# Autodesk Inventor assembly: 20171110 Zusammengesetzt
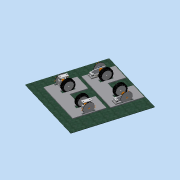
[picture p0: Inventor's stored thumbnail of the model, 180x180]
Saved by Autodesk Inventor 2015 (Build 190159000, 159)
## iProperties
Created: 2017-11-10
Part Number: 20171110 Zusammengesetzt
Document SubType Name: Assembly
Designer: Christoph Soppa
Author: Christoph Soppa
## Documents named in this file (18)
- C:\Users\Christoph Soppa\Desktop\THM Automatisierungs- technik\Sem. 8 Projektarbeit\Bauteile\20171110 Zusammengesetzt.iam
- C:\Users\Christoph Soppa\Desktop\THM Automatisierungs- technik\Sem. 8 Projektarbeit\Bauteile\O Ring 72x3,5x65.ipt
- C:\Users\Christoph Soppa\Desktop\THM Automatisierungs- technik\Sem. 8 Projektarbeit\Bauteile\Rad d72 b4 r3.5.ipt
- C:\Users\Christoph Soppa\Desktop\THM Automatisierungs- technik\Sem. 8 Projektarbeit\Bauteile\Drehgeber 2400 .ipt
- C:\Users\Christoph Soppa\Desktop\THM Automatisierungs- technik\Sem. 8 Projektarbeit\Bauteile\Boden.ipt
- C:\Users\Christoph Soppa\Desktop\THM Automatisierungs- technik\Sem. 8 Projektarbeit\Bauteile\FahrwerkbasisBsp.ipt
- C:\Users\Christoph Soppa\Desktop\THM Automatisierungs- technik\Sem. 8 Projektarbeit\Bauteile\Montageplatte.ipt
- C:\Users\Christoph Soppa\Desktop\THM Automatisierungs- technik\Sem. 8 Projektarbeit\Bauteile\Stehlager 6mm.ipt
- C:\Users\Christoph Soppa\Desktop\THM Automatisierungs- technik\Sem. 8 Projektarbeit\Bauteile\6mm Welle.ipt
- C:\Users\Christoph Soppa\Desktop\THM Automatisierungs- technik\Sem. 8 Projektarbeit\Bauteile\Kupplung.ipt
- C:\Users\Christoph Soppa\Desktop\THM Automatisierungs- technik\Sem. 8 Projektarbeit\Bauteile\Armrechts.ipt
- C:\Users\Christoph Soppa\Desktop\THM Automatisierungs- technik\Sem. 8 Projektarbeit\Bauteile\Armlinks.ipt
- C:\Users\Christoph Soppa\Desktop\THM Automatisierungs- technik\Sem. 8 Projektarbeit\Bauteile\Gummierung Antrieb.ipt
- C:\Users\Christoph Soppa\Desktop\THM Automatisierungs- technik\Sem. 8 Projektarbeit\Bauteile\Antriebsrad 80.ipt
- C:\Users\Christoph Soppa\Desktop\THM Automatisierungs- technik\Sem. 8 Projektarbeit\Bauteile\B Arm.ipt
- C:\Users\Christoph Soppa\Desktop\THM Automatisierungs- technik\Sem. 8 Projektarbeit\Bauteile\B Montageplatte.ipt
- C:\Users\Christoph Soppa\Desktop\THM Automatisierungs- technik\Sem. 8 Projektarbeit\Bauteile\B Oben.ipt
- C:\Users\Christoph Soppa\Desktop\THM Automatisierungs- technik\Sem. 8 Projektarbeit\Bauteile\Federführung.ipt
## Components (47 placed, 17 different names)
1. O Ring 72x3,5x65:1 — Passend:44, Passend:45
2. O Ring 72x3,5x65:2 — Passend:3, Passend:4
3. Rad d72 b4 r3.5:1 — Passend:3, Passend:4, Passend:10, Fluchtend:3, Passend:24, Passend:25, Passend:26
4. Rad d72 b4 r3.5:2 — Passend:40, Passend:41, Passend:42, Passend:45
5. Drehgeber 2400 :1 — Passend:36, Passend:37, Passend:38, Passend:39
6. Drehgeber 2400 :2 — Passend:20, Passend:21, Passend:22, Passend:23
7. Boden:1 — Passend:9, Passend:10, Fluchtend:3, Passend:12, Passend:46, Passend:49, Passend:53, Passend:55, Fluchtend:14, Passend:82, Passend:87, Passend:94, Passend:96
8. FahrwerkbasisBsp:1 — Passend:12, Passend:16, Passend:26, Passend:27, Passend:28, Passend:42, Passend:43, Passend:48, Passend:50, Passend:52, Passend:54
9. Montageplatte:1 — Passend:13, Fluchtend:5, Passend:14, Fluchtend:6, Fluchtend:7, Passend:16
10. Stehlager 6mm:1 — Passend:13, Fluchtend:5, Passend:19
11. Stehlager 6mm:2 — Passend:14, Fluchtend:6, Fluchtend:7, Fluchtend:8, Passend:15, Passend:17
12. 6mm Welle:1 — Fluchtend:8, Passend:15, Passend:18
13. Kupplung:1 — Passend:22, Passend:23, Passend:24, Passend:25, Passend:27
14. Armrechts:1 — Passend:17, Passend:18, Passend:19, Passend:20, Passend:21
15. Stehlager 6mm:3 — Passend:30, Passend:33, Passend:34, Passend:35, Fluchtend:11
16. Stehlager 6mm:4 — Passend:29, Fluchtend:9, Fluchtend:10, Passend:31, Passend:32
17. Montageplatte:2 — Passend:28, Passend:29, Passend:30, Fluchtend:9, Fluchtend:10
18. Armlinks:1 — Passend:31, Passend:32, Passend:33, Passend:34, Passend:36, Passend:37
19. Kupplung:2 — Passend:38, Passend:39, Passend:40, Passend:41, Passend:43, Passend:44, Passend:46
20. 6mm Welle:2 — Passend:35, Fluchtend:11
21. Gummierung Antrieb:1 — Passend:47, Fluchtend:12, Passend:49, Passend:50
22. Gummierung Antrieb:2 — Fluchtend:13, Passend:51, Passend:53, Passend:54
23. Antriebsrad 80:1 — Fluchtend:13, Passend:51, Passend:52
24. Antriebsrad 80:2 — Passend:47, Fluchtend:12, Passend:48
25. FahrwerkbasisBsp:2 — Passend:55, Fluchtend:14, Passend:80, Passend:81, Passend:83, Passend:84, Passend:85, Passend:86, Passend:92, Passend:93, Passend:95, Passend:97
26. B Arm:1 — Passend:67, Passend:68, Passend:71, Passend:72
27. B Montageplatte:1 — Passend:60, Passend:61, Fluchtend:18, Fluchtend:19, Passend:84
28. B Montageplatte:2 — Passend:62, Passend:63, Fluchtend:17, Fluchtend:20, Passend:80
29. B Arm:2 — Passend:66, Passend:69, Passend:70, Passend:73
30. B Oben:1 — Passend:64, Fluchtend:21
31. B Oben:2 — Passend:65, Fluchtend:22
32. Federführung:1 — Passend:63, Fluchtend:20, Passend:64, Fluchtend:21, Passend:67
33. Federführung:2 — Passend:61, Fluchtend:19, Passend:65, Fluchtend:22, Passend:66
34. Federführung:3 — Passend:60, Fluchtend:18, Passend:69
35. Federführung:4 — Passend:62, Fluchtend:17, Passend:68
36. Kupplung:3 — Passend:58, Passend:75, Passend:76, Passend:79, Passend:82, Passend:83
37. Kupplung:4 — Passend:59, Passend:74, Passend:77, Passend:78, Passend:86, Passend:87, Passend:90
38. Drehgeber 2400 :3 — Passend:71, Passend:72, Passend:75, Passend:79
39. Drehgeber 2400 :4 — Passend:70, Passend:73, Passend:74, Passend:78
40. Gummierung Antrieb:3 — Passend:57, Fluchtend:15
41. Gummierung Antrieb:4 — Passend:56, Fluchtend:16, Passend:97
42. O Ring 72x3,5x65:3 — Passend:90, Passend:91
43. O Ring 72x3,5x65:4 — Passend:88, Passend:89
44. Rad d72 b4 r3.5:3 — Passend:59, Passend:77, Passend:85, Passend:91
45. Rad d72 b4 r3.5:4 — Passend:58, Passend:76, Passend:81, Passend:88, Passend:89
46. Antriebsrad 80:3 — Passend:57, Fluchtend:15, Passend:92, Passend:93, Passend:94
47. Antriebsrad 80:4 — Passend:56, Fluchtend:16, Passend:95, Passend:96
## Relationships (109: Mate 90, Flush 19)
- Passend:3 [Mate]: O Ring 72x3,5x65:2 ↔ Rad d72 b4 r3.5:1
- Passend:4 [Mate]: O Ring 72x3,5x65:2 ↔ Rad d72 b4 r3.5:1
- Passend:9 [Mate]: Boden:1
- Passend:10 [Mate] (36 mm): Rad d72 b4 r3.5:1 ↔ Boden:1
- Fluchtend:3 [Flush] (100 mm): Rad d72 b4 r3.5:1 ↔ Boden:1
- Passend:12 [Mate] (5 mm): Boden:1 ↔ FahrwerkbasisBsp:1
- Passend:13 [Mate]: Montageplatte:1 ↔ Stehlager 6mm:1
- Fluchtend:5 [Flush]: Montageplatte:1 ↔ Stehlager 6mm:1
- Passend:14 [Mate]: Montageplatte:1 ↔ Stehlager 6mm:2
- Fluchtend:6 [Flush]: Montageplatte:1 ↔ Stehlager 6mm:2
- Fluchtend:7 [Flush]: Montageplatte:1 ↔ Stehlager 6mm:2
- Fluchtend:8 [Flush]: Stehlager 6mm:2 ↔ 6mm Welle:1
- Passend:15 [Mate]: Stehlager 6mm:2 ↔ 6mm Welle:1
- Passend:16 [Mate]: FahrwerkbasisBsp:1 ↔ Montageplatte:1
- Passend:17 [Mate]: Stehlager 6mm:2 ↔ Armrechts:1
- Passend:18 [Mate]: 6mm Welle:1 ↔ Armrechts:1
- Passend:19 [Mate]: Stehlager 6mm:1 ↔ Armrechts:1
- Passend:20 [Mate]: Drehgeber 2400 :2 ↔ Armrechts:1
- Passend:21 [Mate]: Drehgeber 2400 :2 ↔ Armrechts:1
- Passend:22 [Mate]: Drehgeber 2400 :2 ↔ Kupplung:1
- Passend:23 [Mate]: Drehgeber 2400 :2 ↔ Kupplung:1
- Passend:24 [Mate]: Rad d72 b4 r3.5:1 ↔ Kupplung:1
- Passend:25 [Mate]: Rad d72 b4 r3.5:1 ↔ Kupplung:1
- Passend:26 [Mate] (3 mm): Rad d72 b4 r3.5:1 ↔ FahrwerkbasisBsp:1
- Passend:27 [Mate] (40 mm): FahrwerkbasisBsp:1 ↔ Kupplung:1
- Passend:28 [Mate]: FahrwerkbasisBsp:1 ↔ Montageplatte:2
- Passend:29 [Mate]: Stehlager 6mm:4 ↔ Montageplatte:2
- Passend:30 [Mate]: Stehlager 6mm:3 ↔ Montageplatte:2
- Fluchtend:9 [Flush]: Stehlager 6mm:4 ↔ Montageplatte:2
- Fluchtend:10 [Flush]: Stehlager 6mm:4 ↔ Montageplatte:2
- Passend:31 [Mate]: Stehlager 6mm:4 ↔ Armlinks:1
- Passend:32 [Mate]: Stehlager 6mm:4 ↔ Armlinks:1
- Passend:33 [Mate]: Stehlager 6mm:3 ↔ Armlinks:1
- Passend:34 [Mate]: Stehlager 6mm:3 ↔ Armlinks:1
- Passend:35 [Mate]: Stehlager 6mm:3 ↔ 6mm Welle:2
- Fluchtend:11 [Flush]: Stehlager 6mm:3 ↔ 6mm Welle:2
- Passend:36 [Mate]: Drehgeber 2400 :1 ↔ Armlinks:1
- Passend:37 [Mate]: Drehgeber 2400 :1 ↔ Armlinks:1
- Passend:38 [Mate]: Drehgeber 2400 :1 ↔ Kupplung:2
- Passend:39 [Mate]: Drehgeber 2400 :1 ↔ Kupplung:2
- Passend:40 [Mate]: Rad d72 b4 r3.5:2 ↔ Kupplung:2
- Passend:41 [Mate]: Rad d72 b4 r3.5:2 ↔ Kupplung:2
- Passend:42 [Mate] (3 mm): Rad d72 b4 r3.5:2 ↔ FahrwerkbasisBsp:1
- Passend:43 [Mate] (40 mm): FahrwerkbasisBsp:1 ↔ Kupplung:2
- Passend:44 [Mate]: O Ring 72x3,5x65:1 ↔ Kupplung:2
- Passend:45 [Mate] (-2 mm): O Ring 72x3,5x65:1 ↔ Rad d72 b4 r3.5:2
- Passend:46 [Mate] (36 mm): Boden:1 ↔ Kupplung:2
- Passend:47 [Mate]: Gummierung Antrieb:1 ↔ Antriebsrad 80:2
- Fluchtend:12 [Flush]: Gummierung Antrieb:1 ↔ Antriebsrad 80:2
- Passend:48 [Mate] (2.5 mm): FahrwerkbasisBsp:1 ↔ Antriebsrad 80:2
- Passend:49 [Mate] (40 mm): Boden:1 ↔ Gummierung Antrieb:1
- Passend:50 [Mate] (40 mm): FahrwerkbasisBsp:1 ↔ Gummierung Antrieb:1
- Fluchtend:13 [Flush]: Gummierung Antrieb:2 ↔ Antriebsrad 80:1
- Passend:51 [Mate]: Gummierung Antrieb:2 ↔ Antriebsrad 80:1
- Passend:52 [Mate] (2.5 mm): FahrwerkbasisBsp:1 ↔ Antriebsrad 80:1
- Passend:53 [Mate] (40 mm): Boden:1 ↔ Gummierung Antrieb:2
- Passend:54 [Mate] (40 mm): FahrwerkbasisBsp:1 ↔ Gummierung Antrieb:2
- Passend:55 [Mate] (5 mm): Boden:1 ↔ FahrwerkbasisBsp:2
- Fluchtend:14 [Flush] (100 mm): Boden:1 ↔ FahrwerkbasisBsp:2
- Passend:56 [Mate]: Gummierung Antrieb:4 ↔ Antriebsrad 80:4
- Passend:57 [Mate]: Gummierung Antrieb:3 ↔ Antriebsrad 80:3
- Fluchtend:15 [Flush]: Gummierung Antrieb:3 ↔ Antriebsrad 80:3
- Fluchtend:16 [Flush]: Gummierung Antrieb:4 ↔ Antriebsrad 80:4
- Passend:58 [Mate]: Kupplung:3 ↔ Rad d72 b4 r3.5:4
- Passend:59 [Mate]: Kupplung:4 ↔ Rad d72 b4 r3.5:3
- Passend:60 [Mate]: B Montageplatte:1 ↔ Federführung:3
- Passend:61 [Mate]: B Montageplatte:1 ↔ Federführung:2
- Passend:62 [Mate]: B Montageplatte:2 ↔ Federführung:4
- Passend:63 [Mate]: B Montageplatte:2 ↔ Federführung:1
- Fluchtend:17 [Flush]: B Montageplatte:2 ↔ Federführung:4
- Fluchtend:18 [Flush]: B Montageplatte:1 ↔ Federführung:3
- Fluchtend:19 [Flush]: B Montageplatte:1 ↔ Federführung:2
- Fluchtend:20 [Flush]: B Montageplatte:2 ↔ Federführung:1
- Passend:64 [Mate]: B Oben:1 ↔ Federführung:1
- Fluchtend:21 [Flush]: B Oben:1 ↔ Federführung:1
- Passend:65 [Mate]: B Oben:2 ↔ Federführung:2
- Fluchtend:22 [Flush]: B Oben:2 ↔ Federführung:2
- Passend:66 [Mate]: B Arm:2 ↔ Federführung:2
- Passend:67 [Mate]: B Arm:1 ↔ Federführung:1
- Passend:68 [Mate]: B Arm:1 ↔ Federführung:4
- Passend:69 [Mate]: B Arm:2 ↔ Federführung:3
- Passend:70 [Mate]: B Arm:2 ↔ Drehgeber 2400 :4
- Passend:71 [Mate]: B Arm:1 ↔ Drehgeber 2400 :3
- Passend:72 [Mate]: B Arm:1 ↔ Drehgeber 2400 :3
- Passend:73 [Mate]: B Arm:2 ↔ Drehgeber 2400 :4
- Passend:74 [Mate]: Kupplung:4 ↔ Drehgeber 2400 :4
- Passend:75 [Mate]: Kupplung:3 ↔ Drehgeber 2400 :3
- Passend:76 [Mate]: Kupplung:3 ↔ Rad d72 b4 r3.5:4
- Passend:77 [Mate]: Kupplung:4 ↔ Rad d72 b4 r3.5:3
- Passend:78 [Mate]: Kupplung:4 ↔ Drehgeber 2400 :4
- Passend:79 [Mate]: Kupplung:3 ↔ Drehgeber 2400 :3
- Passend:80 [Mate]: FahrwerkbasisBsp:2 ↔ B Montageplatte:2
- Passend:81 [Mate] (3 mm): FahrwerkbasisBsp:2 ↔ Rad d72 b4 r3.5:4
- Passend:82 [Mate] (36 mm): Boden:1 ↔ Kupplung:3
- Passend:83 [Mate] (40 mm): FahrwerkbasisBsp:2 ↔ Kupplung:3
- Passend:84 [Mate]: FahrwerkbasisBsp:2 ↔ B Montageplatte:1
- Passend:85 [Mate] (3 mm): FahrwerkbasisBsp:2 ↔ Rad d72 b4 r3.5:3
- Passend:86 [Mate] (40 mm): FahrwerkbasisBsp:2 ↔ Kupplung:4
- Passend:87 [Mate] (36 mm): Boden:1 ↔ Kupplung:4
- Passend:88 [Mate]: O Ring 72x3,5x65:4 ↔ Rad d72 b4 r3.5:4
- Passend:89 [Mate] (-2 mm): O Ring 72x3,5x65:4 ↔ Rad d72 b4 r3.5:4
- Passend:90 [Mate]: Kupplung:4 ↔ O Ring 72x3,5x65:3
- Passend:91 [Mate] (-2 mm): O Ring 72x3,5x65:3 ↔ Rad d72 b4 r3.5:3
- Passend:92 [Mate] (2.5 mm): FahrwerkbasisBsp:2 ↔ Antriebsrad 80:3
- Passend:93 [Mate] (40 mm): FahrwerkbasisBsp:2 ↔ Antriebsrad 80:3
- Passend:94 [Mate] (40 mm): Boden:1 ↔ Antriebsrad 80:3
- Passend:95 [Mate] (2.5 mm): FahrwerkbasisBsp:2 ↔ Antriebsrad 80:4
- Passend:96 [Mate] (40 mm): Boden:1 ↔ Antriebsrad 80:4
- Passend:97 [Mate] (40 mm): FahrwerkbasisBsp:2 ↔ Gummierung Antrieb:4
